# Autodesk Inventor assembly: MG_996R
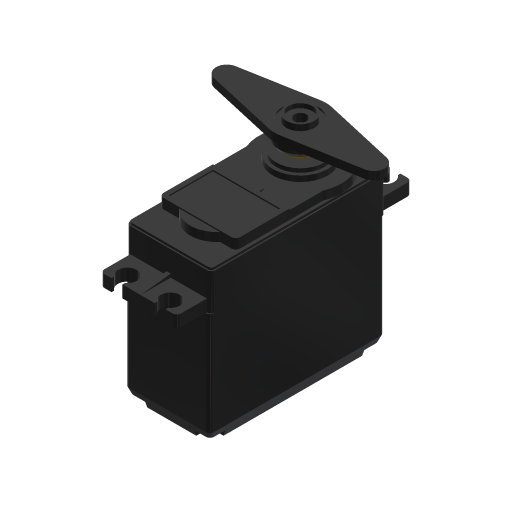
[picture p0: Inventor's stored thumbnail of the model, 512x512]
Saved by Autodesk Inventor 2024 (Build 280153000, 153)
## iProperties
Created: 2016-09-26
Part Number: MG_996R
Document SubType Name: Assembly
Designer: Julian
Author: Julian
## Documents named in this file (6)
- E:\university\大三\大三下\機工實務\圖檔\DesignVer2_encoder\MG996R\MG_996R.iam
- E:\university\大三\大三下\機工實務\圖檔\DesignVer2_encoder\MG996R\Base.ipt
- E:\university\大三\大三下\機工實務\圖檔\DesignVer2_encoder\MG996R\Medio.ipt
- E:\university\大三\大三下\機工實務\圖檔\DesignVer2_encoder\MG996R\Top.ipt
- E:\university\大三\大三下\機工實務\圖檔\DesignVer2_encoder\MG996R\Eje.ipt
- E:\university\大三\大三下\機工實務\圖檔\DesignVer2_encoder\MG996R\Acople circular.ipt
## Components (5 placed, 5 different names)
1. Top:1 — Rígido:2, De rotación:1
2. Medio:1 — Rígido:1, Rígido:2
3. Base:1 — Rígido:1
4. Eje:1 — De rotación:1, De rotación:2
5. Acople circular:1 — De rotación:2
## Relationships (4: WeldJoint 2, RevoluteJoint 2)
- Rígido:1 [WeldJoint]: Medio:1 ↔ Base:1
- Rígido:2 [WeldJoint]: Top:1 ↔ Medio:1
- De rotación:1 [RevoluteJoint]: Top:1 ↔ Eje:1
- De rotación:2 [RevoluteJoint]: Eje:1 ↔ Acople circular:1
